# Autodesk Inventor assembly: XBeeAntennaAssy
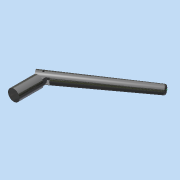
[picture p0: Inventor's stored thumbnail of the model, 180x180]
Saved by Autodesk Inventor 2011 SP1 (Build 150282100, 282)
## iProperties
Created: 2011-08-14
Part Number: XBeeAntennaAssy
Document SubType Name: Assembly
Designer: dgitz
Author: dgitz
## Documents named in this file (3)
- C:\Dropbox\ICARUS\Remote Control Unit (RCU)\RCU v2\Design\Library\XBeeAntennaAssy.iam
- C:\Dropbox\ICARUS\Remote Control Unit (RCU)\RCU v2\Design\Library\XBeeAntenna\AntennaBase.ipt
- C:\Dropbox\ICARUS\Remote Control Unit (RCU)\RCU v2\Design\Library\XBeeAntenna\AntennaMast.ipt
## Components (2 placed, 2 different names)
1. AntennaBase:1 — Angle:1, Mate:1, Mate:2
2. AntennaMast:1 — Angle:1, Mate:1, Mate:2
## Relationships (3: Mate 2, Angle 1)
- Angle:1 (235 deg): AntennaBase:1 ↔ AntennaMast:1
- Mate:1: AntennaBase:1 ↔ AntennaMast:1
- Mate:2 (-0.6604 mm): AntennaBase:1 ↔ AntennaMast:1
